# Autodesk Inventor assembly: 02x01U_2lvl301x01
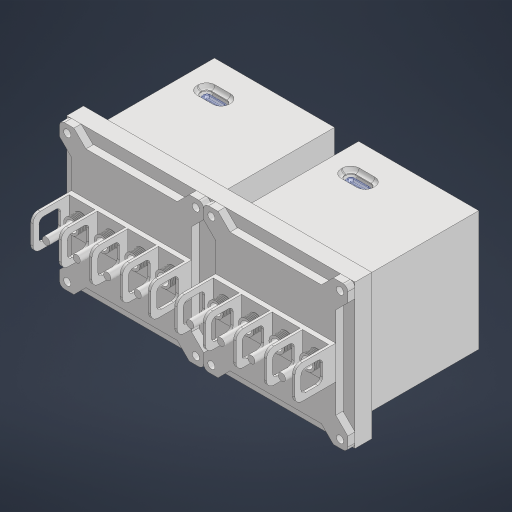
[picture p0: Inventor's stored thumbnail of the model, 512x512]
Saved by Autodesk Inventor 2024 (Build 280153000, 153)
## iProperties
Created: 2026-04-07
Part Number: 02x01U_2lvl301x01
Document SubType Name: Assembly
Designer: schar
Author: schar
## Documents named in this file (3)
- C:\Users\schar\Desktop\MHIPS\models\test_asm\02x01U_2lvl301x01.iam
- C:\Users\schar\Desktop\MHIPS\models\racks\rack_2x1.ipt
- C:\Users\schar\Desktop\MHIPS\models\1x1\1x1_asm_main.iam
## Components (3 placed, 2 different names)
1. rack_2x1:1 — Mate:1, Mate:2, Mate:3, Mate:4, Mate:5, Mate:6
2. 1x1_asm_main:1 [sub-assembly] — Mate:1, Mate:4, Mate:5
3. 1x1_asm_main:2 [sub-assembly] — Mate:2, Mate:3, Mate:6
## Relationships (6: Mate 6)
- Mate:1: rack_2x1:1 ↔ 1x1_asm_main:1
- Mate:2: rack_2x1:1 ↔ 1x1_asm_main:2
- Mate:3: rack_2x1:1 ↔ 1x1_asm_main:2
- Mate:4: rack_2x1:1 ↔ 1x1_asm_main:1
- Mate:5: rack_2x1:1 ↔ 1x1_asm_main:1
- Mate:6: rack_2x1:1 ↔ 1x1_asm_main:2
